# Autodesk Inventor assembly: robot
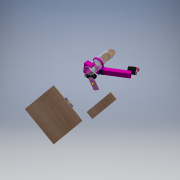
[picture p0: Inventor's stored thumbnail of the model, 180x180]
Saved by Autodesk Inventor 2017 (Build 210142000, 142)
## iProperties
Created: 2018-04-01
Part Number: robot
Document SubType Name: Assembly
Designer: franc
Author: franc
## Documents named in this file (5)
- C:\Users\franc\Desktop\EsialRobotik\Mecanique\2018\robot\robot.iam
- C:\Users\franc\Desktop\EsialRobotik\Mecanique\base_roulante\baseRoulante.iam
- C:\Users\franc\Desktop\EsialRobotik\Mecanique\2018\robot\socle-robot.ipt
- C:\Users\franc\Desktop\EsialRobotik\Mecanique\2018\robot\traitement-eau\recuperation.iam
- C:\Users\franc\Desktop\EsialRobotik\Mecanique\2018\robot\etage-bras.ipt
## Components (4 placed, 4 different names)
1. baseRoulante:1 [sub-assembly] — Affleurement:1, Affleurement:2, Placage:1, Angle:1, Placage:2
2. socle-robot:1 — Affleurement:1, Affleurement:2, Placage:1, Affleurement:3
3. etage-bras:1 — Affleurement:3, Angle:1
4. recuperation:1 [sub-assembly] — Placage:2
## Relationships (6: Flush 3, Mate 2, Angle 1)
- Affleurement:1 [Flush] (5 mm): baseRoulante:1 ↔ socle-robot:1
- Affleurement:2 [Flush] (54 mm): baseRoulante:1 ↔ socle-robot:1
- Placage:1 [Mate]: baseRoulante:1 ↔ socle-robot:1
- Affleurement:3 [Flush] (5 mm): socle-robot:1 ↔ etage-bras:1
- Angle:1 (0 deg): baseRoulante:1 ↔ etage-bras:1
- Placage:2 [Mate] (93 mm): baseRoulante:1 ↔ recuperation:1
